# Autodesk Inventor assembly: robot_solid
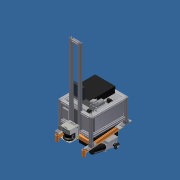
[picture p0: Inventor's stored thumbnail of the model, 180x180]
Saved by Autodesk Inventor 2012 (Build 160160000, 160)
## iProperties
Created: 2012-03-08
Part Number: robot_solid
Document SubType Name: Assembly
Designer: esv
Mass: 186693 g
Surface Area: 125384 cm^2
Volume: 159546 cm^3
Density: 1.17015 g/cm^3
Author: esv
## Documents named in this file (16)
- C:\Users\Edward\Documents\masters\CAD\robot_solid.iam
- C:\Users\Edward\Documents\masters\CAD\Frame\frame bracket.ipt
- C:\Users\Edward\Documents\masters\CAD\IRC5\IRC5_Compact.ipt
- C:\Users\Edward\Documents\masters\CAD\PC\PC.ipt
- C:\Users\Edward\Documents\masters\CAD\SICK\SICK LMS291.ipt
- C:\Users\Edward\Documents\masters\CAD\Frame\back frame plate.ipt
- C:\Users\Edward\Documents\masters\CAD\Frame\front frame plate.ipt
- C:\Users\Edward\Documents\masters\CAD\Frame\top plate.ipt
- C:\Users\Edward\Documents\masters\CAD\Pneumatics\compressor\compressor.iam
- C:\Users\Edward\Documents\masters\CAD\Spike\Spike H.iam
- C:\Users\Edward\Documents\masters\CAD\Breaker\Breaker.iam
- C:\Users\Edward\Documents\masters\CAD\Router\router keepout.ipt
- C:\Users\Edward\Documents\masters\CAD\Frame\short frame bracket.ipt
- C:\Users\Edward\Documents\masters\CAD\base plate.iam
- C:\Users\Edward\Documents\masters\CAD\al_frame.iam
- C:\Users\Edward\Documents\masters\CAD\Invacare\frame_solid.iam
## Components (19 placed, 15 different names)
1. frame bracket:1 — Flush:5, Mate:72, Flush:56, Mate:74, Mate:132
2. frame bracket:4 — Flush:5, Flush:57, Mate:75, Mate:76
3. frame_solid:1 [sub-assembly] — Mate:17, Tangent:8, Mate:137, Flush:99
4. IRC5_Compact:1 — Flush:2, Mate:122, Mate:126
5. PC:1 — Mate:36, Flush:63, Flush:91
6. SICK LMS291:1 — Mate:118, Insert:12
7. back frame plate:1 — Flush:82, Insert:7, Flush:88, Flush:89, Flush:96, Flush:99
8. back frame plate:2 — Insert:6, Flush:87, Flush:88, Flush:90, Flush:98
9. front frame plate:1 — Flush:57, Mate:75, Mate:76, Flush:89, Tangent:8, Flush:96, Flush:97, Mate:137
10. front frame plate:2 — Mate:72, Flush:56, Mate:74, Flush:90, Flush:97, Flush:98
11. top plate:1 — Mate:36, Mate:80, Flush:63, Mate:81, Insert:1, Insert:2, Insert:3, Mate:82, Insert:4, Insert:5, Flush:64, Mate:121, Flush:85, Flush:86, Flush:91
12. compressor:1 [sub-assembly] — Mate:80, Insert:2, Insert:3
13. Spike H:1 [sub-assembly] — Mate:81, Insert:1
14. Breaker:1 [sub-assembly] — Mate:82, Insert:4, Insert:5
15. router keepout:1 — Flush:64, Mate:83, Mate:119
16. short frame bracket:1 — Insert:6, Flush:87, Mate:127, Mate:129, Mate:130
17. short frame bracket:2 — Flush:82, Insert:7, Mate:131
18. base plate:1 [sub-assembly] — Mate:123, Mate:124, Mate:125, Mate:126
19. al_frame:1 [sub-assembly] — Mate:119, Mate:121, Flush:85, Flush:86, Mate:122, Insert:12, Mate:123, Mate:124, Mate:125, Mate:127, Mate:129, Mate:130, Mate:131, Mate:132
## Relationships (53: Mate 25, Flush 19, Insert 8, Tangent 1)
- Flush:2 (-225 mm): IRC5_Compact:1
- Flush:5: frame bracket:1 ↔ frame bracket:4
- Mate:17: frame_solid:1
- Mate:36: PC:1 ↔ top plate:1
- Flush:40 (-368.3 mm)
- Mate:56
- Mate:72: frame bracket:1 ↔ front frame plate:2
- Flush:56: frame bracket:1 ↔ front frame plate:2
- Mate:74: frame bracket:1 ↔ front frame plate:2
- Flush:57: frame bracket:4 ↔ front frame plate:1
- Mate:75: frame bracket:4 ↔ front frame plate:1
- Mate:76: frame bracket:4 ↔ front frame plate:1
- Mate:80: top plate:1 ↔ compressor:1
- Flush:63 (-50.8 mm): PC:1 ↔ top plate:1
- Mate:81: top plate:1 ↔ Spike H:1
- Insert:1: top plate:1 ↔ Spike H:1
- Insert:2: top plate:1 ↔ compressor:1
- Insert:3: top plate:1 ↔ compressor:1
- Mate:82: top plate:1 ↔ Breaker:1
- Insert:4: top plate:1 ↔ Breaker:1
- Insert:5: top plate:1 ↔ Breaker:1
- Flush:64 (-304.8 mm): top plate:1 ↔ router keepout:1
- Mate:83: router keepout:1
- Insert:6: back frame plate:2 ↔ short frame bracket:1
- Flush:82: back frame plate:1 ↔ short frame bracket:2
- Insert:7: back frame plate:1 ↔ short frame bracket:2
- Mate:118: SICK LMS291:1
- Mate:119: router keepout:1 ↔ al_frame:1
- Mate:121: top plate:1 ↔ al_frame:1
- Flush:85: top plate:1 ↔ al_frame:1
- Flush:86: top plate:1 ↔ al_frame:1
- Mate:122: IRC5_Compact:1 ↔ al_frame:1
- Insert:12: SICK LMS291:1 ↔ al_frame:1
- Mate:123: base plate:1 ↔ al_frame:1
- Mate:124: base plate:1 ↔ al_frame:1
- Mate:125: base plate:1 ↔ al_frame:1
- Mate:126: IRC5_Compact:1 ↔ base plate:1
- Flush:87: back frame plate:2 ↔ short frame bracket:1
- Flush:88: back frame plate:1 ↔ back frame plate:2
- Flush:89: back frame plate:1 ↔ front frame plate:1
- Flush:90: back frame plate:2 ↔ front frame plate:2
- Mate:127: short frame bracket:1 ↔ al_frame:1
- Mate:129: short frame bracket:1 ↔ al_frame:1
- Mate:130: short frame bracket:1 ↔ al_frame:1
- Mate:131: short frame bracket:2 ↔ al_frame:1
- Flush:91 (50.8 mm): PC:1 ↔ top plate:1
- Mate:132: frame bracket:1 ↔ al_frame:1
- Tangent:8: frame_solid:1 ↔ front frame plate:1
- Flush:96: back frame plate:1 ↔ front frame plate:1
- Flush:97: front frame plate:1 ↔ front frame plate:2
- Flush:98: back frame plate:2 ↔ front frame plate:2
- Mate:137: frame_solid:1 ↔ front frame plate:1
- Flush:99 (88.9 mm): frame_solid:1 ↔ back frame plate:1
